# Autodesk Inventor assembly: centre wing
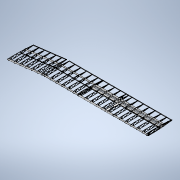
[picture p0: Inventor's stored thumbnail of the model, 180x180]
Saved by Autodesk Inventor 2022 (Build 260153000, 153)
## iProperties
Created: 2021-03-09
Part Number: centre wing
Document SubType Name: Assembly
Designer: Ferdinand Hubbard
Author: Ferdinand Hubbard
## Documents named in this file (20)
- C:\Users\Ferdinand Hubbard\Desktop\solarplane\cad\right wing section.iam
- C:\Users\Ferdinand Hubbard\Desktop\solarplane\cad\tubes\normal tubes\15mm tube.ipt
- C:\Users\Ferdinand Hubbard\Desktop\solarplane\cad\tubes\normal tubes\18mm tube.ipt
- C:\Users\Ferdinand Hubbard\Desktop\solarplane\cad\airfoils\full airfoil\full airfoil blueprint 16 mm.ipt
- C:\Users\Ferdinand Hubbard\Desktop\solarplane\cad\airfoils\full airfoil adjacent to aileron\full adjacent to aileron airfoil 16 mm big hole.ipt
- C:\Users\Ferdinand Hubbard\Desktop\solarplane\cad\airfoils\front half aileron\front half airfoil 19 mm.ipt
- C:\Users\Ferdinand Hubbard\Desktop\solarplane\cad\airfoils\back half aileron\back half aileron airfoil 19mm.ipt
- C:\Users\Ferdinand Hubbard\Desktop\solarplane\cad\tubes\normal tubes\7mm tube.ipt
- C:\Users\Ferdinand Hubbard\Desktop\solarplane\cad\tubes\normal tubes\straight connector aileron spar.ipt
- C:\Users\Ferdinand Hubbard\Desktop\solarplane\cad\airfoils\front half aileron\front half airfoil 16 mm.ipt
- C:\Users\Ferdinand Hubbard\Desktop\solarplane\cad\tubes\normal tubes\angle connector 16 mm.ipt
- C:\Users\Ferdinand Hubbard\Desktop\solarplane\cad\tubes\back aileron tubes\15mm tube.ipt
- C:\Users\Ferdinand Hubbard\Desktop\solarplane\cad\tubes\back aileron tubes\18mm tube.ipt
- C:\Users\Ferdinand Hubbard\Desktop\solarplane\cad\tubes\pre-aileron tubes\angle connector 16 mm.ipt
- C:\Users\Ferdinand Hubbard\Desktop\solarplane\cad\wood spars\wood 5 5 476.ipt
- C:\Users\Ferdinand Hubbard\Desktop\solarplane\cad\wood spars\wood 5 5 478.ipt
- C:\Users\Ferdinand Hubbard\Desktop\solarplane\cad\wood spars\wood 5 5 1459.ipt
- C:\Users\Ferdinand Hubbard\Desktop\solarplane\cad\wood spars\wood 5 5 968.ipt
- C:\Users\Ferdinand Hubbard\Desktop\solarplane\cad\servo mount.ipt
- C:\Users\Ferdinand Hubbard\Desktop\solarplane\cad\aileron arm mount.ipt
## Components (65 placed, 16 different names)
1. angle connector 16 mm:7 — Mate:1, Mate:2, Mate:3, Mate:4, Angle:3
2. angle connector 16 mm:4 — Angle:5, Mate:107
3. 15mm tube:1 — Mate:1, Mate:2, Flush:1, Mate:32, Angle:2, Flush:4, Flush:10
4. 15mm tube:5 — Angle:6, Mate:50, Flush:12, Mate:107, Flush:16
5. 15mm tube:2 — Mate:3, Mate:4, Mate:5, Mate:6, Mate:49, Angle:4
6. 15mm tube:3 — Mate:7, Mate:8, Mate:145
7. 18mm tube:1 — Mate:5, Mate:6, Mate:7, Mate:8, Mate:210
8. full airfoil blueprint 16 mm:1 — Mate:9, Mate:10, Mate:11, Flush:1, Mate:32, Mate:33, Flush:2, Angle:1, Angle:2, Flush:22, Flush:23, Flush:24, Mate:196, Mate:197, Mate:198, Mate:199, Mate:200, Mate:201
9. full airfoil blueprint 16 mm:2 — Mate:9, Mate:10, Mate:11, Mate:15, Mate:16, Mate:17
10. full airfoil blueprint 16 mm:3 — Mate:15, Mate:16, Mate:17
11. full airfoil blueprint 16 mm:4 — Mate:21, Mate:22, Mate:23
12. full airfoil blueprint 16 mm:5 — Mate:21, Mate:22, Mate:23
13. full airfoil blueprint 16 mm:6 — Mate:91, Mate:92
14. 15mm tube:4 — Mate:33, Flush:2, Angle:1, Flush:4, Flush:9
15. full airfoil blueprint 16 mm:7 — Mate:49, Angle:3, Angle:4, Angle:5, Angle:6, Mate:50, Flush:16, Flush:25, Mate:202, Mate:203
16. full airfoil blueprint 16 mm:8
17. full airfoil blueprint 16 mm:9
18. full airfoil blueprint 16 mm:10
19. full airfoil blueprint 16 mm:11 — Mate:93, Flush:11, Mate:104, Mate:105, Mate:106
20. full airfoil blueprint 16 mm:20 — Mate:91, Mate:92, Flush:9, Flush:10
21. full adjacent to aileron airfoil 16 mm big hole:1 — Mate:93, Flush:11, Flush:12, Mate:94, Mate:96, Flush:13, Mate:97, Angle:7, Flush:14, Mate:103, Mate:108, Flush:20, Mate:187, Mate:191, Angle:9
22. front half airfoil 19 mm:1 — Mate:94, Mate:103, Mate:109, Mate:110, Mate:111, Mate:191
23. back half aileron airfoil 19mm:1 — Mate:96, Flush:13, Angle:8, Mate:98, Mate:108, Flush:17, Mate:150, Mate:181, Mate:182
24. 7mm tube:1 — Angle:7, Mate:97, Flush:14, Mate:99, Mate:100, Mate:212
25. 18mm tube:4 — Angle:8, Mate:98, Flush:17, Mate:148, Mate:149, Mate:213
26. straight connector aileron spar:1 — Mate:99, Mate:100, Mate:101, Mate:102
27. 7mm tube:2 — Mate:101, Mate:102, Mate:147
28. full airfoil blueprint 16 mm:21 — Mate:104, Mate:105, Mate:106
29. front half airfoil 19 mm:2 — Mate:109, Mate:110, Mate:111, Mate:115, Mate:116, Mate:117
30. front half airfoil 19 mm:3 — Mate:115, Mate:116, Mate:117
31. front half airfoil 19 mm:4 — Mate:124, Mate:125, Mate:126
32. 18mm tube:3 — Flush:20, Mate:186, Mate:187, Angle:9, Mate:211
33. 15mm tube:6 — Flush:19, Mate:186, Mate:188
34. front half airfoil 19 mm:5 — Mate:124, Mate:125, Mate:126
35. front half airfoil 19 mm:6 — Mate:136, Mate:189, Mate:190
36. front half airfoil 16 mm:1 — Mate:127, Mate:128, Mate:129, Mate:136, Mate:189, Mate:190
37. front half airfoil 16 mm:2 — Mate:127, Mate:128, Mate:129, Mate:133, Mate:134, Mate:135
38. front half airfoil 16 mm:3 — Mate:133, Mate:134, Mate:135
39. front half airfoil 16 mm:4 — Mate:142, Mate:143, Mate:144
40. front half airfoil 16 mm:5 — Mate:142, Mate:143, Mate:144
41. front half airfoil 16 mm:6 — Mate:194, Mate:195
42. full adjacent to aileron airfoil 16 mm big hole:2 — Mate:145, Mate:147, Flush:19, Mate:185, Mate:188, Mate:192, Flush:26, Flush:27, Mate:204, Mate:205, Mate:206, Mate:207
43. 15mm tube:7 — Mate:148, Mate:149, Flush:21
44. back half aileron airfoil 19mm:2 — Mate:150, Mate:151, Mate:152, Mate:153, Mate:181, Mate:182
45. back half aileron airfoil 19mm:3 — Mate:151, Mate:152, Mate:153, Mate:157, Mate:158, Mate:159
46. back half aileron airfoil 19mm:4 — Mate:157, Mate:158, Mate:159
47. back half aileron airfoil 19mm:5 — Mate:169, Mate:170, Mate:171
48. back half aileron airfoil 19mm:6 — Mate:169, Mate:170, Mate:171
49. back half aileron airfoil 19mm:7
50. back half aileron airfoil 19mm:8
51. back half aileron airfoil 19mm:9 — Mate:178, Mate:179, Mate:180
52. back half aileron airfoil 19mm:10 — Mate:178, Mate:179, Mate:180
53. back half aileron airfoil 19mm:11
54. back half aileron airfoil 19mm:12 — Mate:183, Mate:184
55. back half aileron airfoil 19mm:13 — Flush:21, Mate:183, Mate:184, Mate:185, Flush:28, Mate:208, Mate:209
56. front half airfoil 16 mm:7 — Mate:192, Mate:194, Mate:195
57. wood 5 5 476:1 — Flush:24, Mate:200, Mate:201
58. wood 5 5 476:2 — Flush:23, Mate:198, Mate:199
59. wood 5 5 476:3 — Flush:22, Mate:196, Mate:197
60. wood 5 5 478:1 — Flush:25, Mate:202, Mate:203
61. wood 5 5 1459:1 — Flush:27, Mate:206, Mate:207
62. wood 5 5 1459:2 — Flush:26, Mate:204, Mate:205
63. wood 5 5 968:1 — Flush:28, Mate:208, Mate:209
64. servo mount:1 — Mate:210, Mate:211, Mate:214
65. aileron arm mount:1 — Mate:212, Mate:213, Mate:214
## Relationships (188: Mate 158, Flush 21, Angle 9)
- Mate:1: angle connector 16 mm:7 ↔ 15mm tube:1
- Mate:2: angle connector 16 mm:7 ↔ 15mm tube:1
- Mate:3: angle connector 16 mm:7 ↔ 15mm tube:2
- Mate:4: angle connector 16 mm:7 ↔ 15mm tube:2
- Mate:5: 15mm tube:2 ↔ 18mm tube:1
- Mate:6: 15mm tube:2 ↔ 18mm tube:1
- Mate:7: 15mm tube:3 ↔ 18mm tube:1
- Mate:8: 15mm tube:3 ↔ 18mm tube:1
- Mate:9 (80 mm): full airfoil blueprint 16 mm:1 ↔ full airfoil blueprint 16 mm:2
- Mate:10: full airfoil blueprint 16 mm:1 ↔ full airfoil blueprint 16 mm:2
- Mate:11: full airfoil blueprint 16 mm:1 ↔ full airfoil blueprint 16 mm:2
- [Mate] (80 mm): full airfoil blueprint 16 mm:3 ↔ full airfoil blueprint 16 mm:4
- [Mate]: full airfoil blueprint 16 mm:3 ↔ full airfoil blueprint 16 mm:4
- [Mate]: full airfoil blueprint 16 mm:3 ↔ full airfoil blueprint 16 mm:4
- Mate:15: full airfoil blueprint 16 mm:2 ↔ full airfoil blueprint 16 mm:3
- Mate:16: full airfoil blueprint 16 mm:2 ↔ full airfoil blueprint 16 mm:3
- Mate:17 (80 mm): full airfoil blueprint 16 mm:2 ↔ full airfoil blueprint 16 mm:3
- Flush:1 (12 mm): 15mm tube:1 ↔ full airfoil blueprint 16 mm:1
- [Mate] (80 mm): full airfoil blueprint 16 mm:5 ↔ full airfoil blueprint 16 mm:6
- [Mate]: full airfoil blueprint 16 mm:5 ↔ full airfoil blueprint 16 mm:6
- [Mate]: full airfoil blueprint 16 mm:5 ↔ full airfoil blueprint 16 mm:6
- Mate:21 (80 mm): full airfoil blueprint 16 mm:4 ↔ full airfoil blueprint 16 mm:5
- Mate:22: full airfoil blueprint 16 mm:4 ↔ full airfoil blueprint 16 mm:5
- Mate:23: full airfoil blueprint 16 mm:4 ↔ full airfoil blueprint 16 mm:5
- [Mate]: angle connector 16 mm:4 ↔ 15mm tube:4
- [Mate]: angle connector 16 mm:4 ↔ 15mm tube:4
- Mate:32: 15mm tube:1 ↔ full airfoil blueprint 16 mm:1
- Mate:33: full airfoil blueprint 16 mm:1 ↔ 15mm tube:4
- Flush:2 (12 mm): full airfoil blueprint 16 mm:1 ↔ 15mm tube:4
- [Mate] (80 mm): full airfoil blueprint 16 mm:7 ↔ full airfoil blueprint 16 mm:8
- [Mate]: full airfoil blueprint 16 mm:7 ↔ full airfoil blueprint 16 mm:8
- [Mate]: full airfoil blueprint 16 mm:7 ↔ full airfoil blueprint 16 mm:8
- [Mate] (80 mm): full airfoil blueprint 16 mm:9 ↔ full airfoil blueprint 16 mm:10
- [Mate]: full airfoil blueprint 16 mm:9 ↔ full airfoil blueprint 16 mm:10
- [Mate]: full airfoil blueprint 16 mm:9 ↔ full airfoil blueprint 16 mm:10
- [Mate]: full airfoil blueprint 16 mm:8 ↔ full airfoil blueprint 16 mm:9
- [Mate]: full airfoil blueprint 16 mm:8 ↔ full airfoil blueprint 16 mm:9
- [Mate] (80 mm): full airfoil blueprint 16 mm:8 ↔ full airfoil blueprint 16 mm:9
- [Mate] (80 mm): full airfoil blueprint 16 mm:10 ↔ full airfoil blueprint 16 mm:11
- [Mate]: full airfoil blueprint 16 mm:10 ↔ full airfoil blueprint 16 mm:11
- [Mate]: full airfoil blueprint 16 mm:10 ↔ full airfoil blueprint 16 mm:11
- Angle:1 (270 deg): full airfoil blueprint 16 mm:1 ↔ 15mm tube:4
- Angle:2 (270 deg): 15mm tube:1 ↔ full airfoil blueprint 16 mm:1
- Mate:49: 15mm tube:2 ↔ full airfoil blueprint 16 mm:7
- Flush:4: 15mm tube:1 ↔ 15mm tube:4
- Angle:3 (0 deg): angle connector 16 mm:7 ↔ full airfoil blueprint 16 mm:7
- Angle:4 (180 deg): 15mm tube:2 ↔ full airfoil blueprint 16 mm:7
- Angle:5 (0 deg): angle connector 16 mm:4 ↔ full airfoil blueprint 16 mm:7
- Angle:6 (0 deg): 15mm tube:5 ↔ full airfoil blueprint 16 mm:7
- Mate:50: 15mm tube:5 ↔ full airfoil blueprint 16 mm:7
- Mate:91: full airfoil blueprint 16 mm:6 ↔ full airfoil blueprint 16 mm:20
- Mate:92: full airfoil blueprint 16 mm:6 ↔ full airfoil blueprint 16 mm:20
- Flush:9 (12 mm): 15mm tube:4 ↔ full airfoil blueprint 16 mm:20
- Flush:10 (12 mm): 15mm tube:1 ↔ full airfoil blueprint 16 mm:20
- Mate:93: full airfoil blueprint 16 mm:11 ↔ full adjacent to aileron airfoil 16 mm big hole:1
- Flush:11: full airfoil blueprint 16 mm:11 ↔ full adjacent to aileron airfoil 16 mm big hole:1
- Flush:12: 15mm tube:5 ↔ full adjacent to aileron airfoil 16 mm big hole:1
- Mate:94: full adjacent to aileron airfoil 16 mm big hole:1 ↔ front half airfoil 19 mm:1
- Mate:96: full adjacent to aileron airfoil 16 mm big hole:1 ↔ back half aileron airfoil 19mm:1
- Flush:13: full adjacent to aileron airfoil 16 mm big hole:1 ↔ back half aileron airfoil 19mm:1
- Angle:7 (0 deg): full adjacent to aileron airfoil 16 mm big hole:1 ↔ 7mm tube:1
- Mate:97: full adjacent to aileron airfoil 16 mm big hole:1 ↔ 7mm tube:1
- Angle:8 (0 deg): back half aileron airfoil 19mm:1 ↔ 18mm tube:4
- Mate:98: back half aileron airfoil 19mm:1 ↔ 18mm tube:4
- Flush:14 (8 mm): full adjacent to aileron airfoil 16 mm big hole:1 ↔ 7mm tube:1
- Mate:99: 7mm tube:1 ↔ straight connector aileron spar:1
- Mate:100: 7mm tube:1 ↔ straight connector aileron spar:1
- Mate:101: straight connector aileron spar:1 ↔ 7mm tube:2
- Mate:102: straight connector aileron spar:1 ↔ 7mm tube:2
- Mate:103 (12 mm): full adjacent to aileron airfoil 16 mm big hole:1 ↔ front half airfoil 19 mm:1
- Mate:104 (80 mm): full airfoil blueprint 16 mm:11 ↔ full airfoil blueprint 16 mm:21
- Mate:105: full airfoil blueprint 16 mm:11 ↔ full airfoil blueprint 16 mm:21
- Mate:106: full airfoil blueprint 16 mm:11 ↔ full airfoil blueprint 16 mm:21
- Mate:107: angle connector 16 mm:4 ↔ 15mm tube:5
- Flush:16 (22 mm): 15mm tube:5 ↔ full airfoil blueprint 16 mm:7
- Mate:108 (4 mm): full adjacent to aileron airfoil 16 mm big hole:1 ↔ back half aileron airfoil 19mm:1
- Flush:17 (1 mm): back half aileron airfoil 19mm:1 ↔ 18mm tube:4
- Mate:109 (80 mm): front half airfoil 19 mm:1 ↔ front half airfoil 19 mm:2
- Mate:110: front half airfoil 19 mm:1 ↔ front half airfoil 19 mm:2
- Mate:111: front half airfoil 19 mm:1 ↔ front half airfoil 19 mm:2
- [Mate] (80 mm): front half airfoil 19 mm:3 ↔ front half airfoil 19 mm:4
- [Mate]: front half airfoil 19 mm:3 ↔ front half airfoil 19 mm:4
- [Mate]: front half airfoil 19 mm:3 ↔ front half airfoil 19 mm:4
- Mate:115 (80 mm): front half airfoil 19 mm:2 ↔ front half airfoil 19 mm:3
- Mate:116: front half airfoil 19 mm:2 ↔ front half airfoil 19 mm:3
- Mate:117: front half airfoil 19 mm:2 ↔ front half airfoil 19 mm:3
- [Mate]: 18mm tube:3 ↔ 15mm tube:6
- [Mate] (80 mm): front half airfoil 19 mm:5 ↔ front half airfoil 19 mm:6
- [Mate]: front half airfoil 19 mm:5 ↔ front half airfoil 19 mm:6
- [Mate]: front half airfoil 19 mm:5 ↔ front half airfoil 19 mm:6
- Mate:124 (80 mm): front half airfoil 19 mm:4 ↔ front half airfoil 19 mm:5
- Mate:125: front half airfoil 19 mm:4 ↔ front half airfoil 19 mm:5
- Mate:126: front half airfoil 19 mm:4 ↔ front half airfoil 19 mm:5
- Mate:127 (80 mm): front half airfoil 16 mm:1 ↔ front half airfoil 16 mm:2
- Mate:128: front half airfoil 16 mm:1 ↔ front half airfoil 16 mm:2
- Mate:129: front half airfoil 16 mm:1 ↔ front half airfoil 16 mm:2
- [Mate] (80 mm): front half airfoil 16 mm:3 ↔ front half airfoil 16 mm:4
- [Mate]: front half airfoil 16 mm:3 ↔ front half airfoil 16 mm:4
- [Mate]: front half airfoil 16 mm:3 ↔ front half airfoil 16 mm:4
- Mate:133 (80 mm): front half airfoil 16 mm:2 ↔ front half airfoil 16 mm:3
- Mate:134: front half airfoil 16 mm:2 ↔ front half airfoil 16 mm:3
- Mate:135: front half airfoil 16 mm:2 ↔ front half airfoil 16 mm:3
- Mate:136 (80 mm): front half airfoil 19 mm:6 ↔ front half airfoil 16 mm:1
- [Mate] (80 mm): front half airfoil 16 mm:5 ↔ front half airfoil 16 mm:6
- [Mate]: front half airfoil 16 mm:5 ↔ front half airfoil 16 mm:6
- [Mate]: front half airfoil 16 mm:5 ↔ front half airfoil 16 mm:6
- Mate:142 (80 mm): front half airfoil 16 mm:4 ↔ front half airfoil 16 mm:5
- Mate:143: front half airfoil 16 mm:4 ↔ front half airfoil 16 mm:5
- Mate:144: front half airfoil 16 mm:4 ↔ front half airfoil 16 mm:5
- Mate:145: 15mm tube:3 ↔ full adjacent to aileron airfoil 16 mm big hole:2
- Mate:147: 7mm tube:2 ↔ full adjacent to aileron airfoil 16 mm big hole:2
- Mate:148: 18mm tube:4 ↔ 15mm tube:7
- Mate:149: 18mm tube:4 ↔ 15mm tube:7
- Flush:19 (1 mm): 15mm tube:6 ↔ full adjacent to aileron airfoil 16 mm big hole:2
- Mate:150 (80 mm): back half aileron airfoil 19mm:1 ↔ back half aileron airfoil 19mm:2
- Mate:151 (80 mm): back half aileron airfoil 19mm:2 ↔ back half aileron airfoil 19mm:3
- Mate:152: back half aileron airfoil 19mm:2 ↔ back half aileron airfoil 19mm:3
- Mate:153: back half aileron airfoil 19mm:2 ↔ back half aileron airfoil 19mm:3
- [Mate] (80 mm): back half aileron airfoil 19mm:4 ↔ back half aileron airfoil 19mm:5
- [Mate]: back half aileron airfoil 19mm:4 ↔ back half aileron airfoil 19mm:5
- [Mate]: back half aileron airfoil 19mm:4 ↔ back half aileron airfoil 19mm:5
- Mate:157: back half aileron airfoil 19mm:3 ↔ back half aileron airfoil 19mm:4
- Mate:158 (80 mm): back half aileron airfoil 19mm:3 ↔ back half aileron airfoil 19mm:4
- Mate:159: back half aileron airfoil 19mm:3 ↔ back half aileron airfoil 19mm:4
- [Mate] (80 mm): back half aileron airfoil 19mm:6 ↔ back half aileron airfoil 19mm:7
- [Mate]: back half aileron airfoil 19mm:6 ↔ back half aileron airfoil 19mm:7
- [Mate]: back half aileron airfoil 19mm:6 ↔ back half aileron airfoil 19mm:7
- [Mate] (80 mm): back half aileron airfoil 19mm:8 ↔ back half aileron airfoil 19mm:9
- [Mate]: back half aileron airfoil 19mm:8 ↔ back half aileron airfoil 19mm:9
- [Mate]: back half aileron airfoil 19mm:8 ↔ back half aileron airfoil 19mm:9
- [Mate]: back half aileron airfoil 19mm:7 ↔ back half aileron airfoil 19mm:8
- [Mate] (80 mm): back half aileron airfoil 19mm:7 ↔ back half aileron airfoil 19mm:8
- [Mate]: back half aileron airfoil 19mm:7 ↔ back half aileron airfoil 19mm:8
- Mate:169 (80 mm): back half aileron airfoil 19mm:5 ↔ back half aileron airfoil 19mm:6
- Mate:170: back half aileron airfoil 19mm:5 ↔ back half aileron airfoil 19mm:6
- Mate:171: back half aileron airfoil 19mm:5 ↔ back half aileron airfoil 19mm:6
- [Mate] (80 mm): back half aileron airfoil 19mm:11 ↔ back half aileron airfoil 19mm:12
- [Mate]: back half aileron airfoil 19mm:11 ↔ back half aileron airfoil 19mm:12
- [Mate]: back half aileron airfoil 19mm:11 ↔ back half aileron airfoil 19mm:12
- [Mate]: back half aileron airfoil 19mm:10 ↔ back half aileron airfoil 19mm:11
- [Mate] (80 mm): back half aileron airfoil 19mm:10 ↔ back half aileron airfoil 19mm:11
- [Mate]: back half aileron airfoil 19mm:10 ↔ back half aileron airfoil 19mm:11
- Mate:178 (80 mm): back half aileron airfoil 19mm:9 ↔ back half aileron airfoil 19mm:10
- Mate:179: back half aileron airfoil 19mm:9 ↔ back half aileron airfoil 19mm:10
- Mate:180: back half aileron airfoil 19mm:9 ↔ back half aileron airfoil 19mm:10
- Mate:181: back half aileron airfoil 19mm:1 ↔ back half aileron airfoil 19mm:2
- Mate:182: back half aileron airfoil 19mm:1 ↔ back half aileron airfoil 19mm:2
- Flush:21 (1 mm): 15mm tube:7 ↔ back half aileron airfoil 19mm:13
- Mate:183: back half aileron airfoil 19mm:12 ↔ back half aileron airfoil 19mm:13
- Mate:184: back half aileron airfoil 19mm:12 ↔ back half aileron airfoil 19mm:13
- Flush:20 (1 mm): full adjacent to aileron airfoil 16 mm big hole:1 ↔ 18mm tube:3
- Mate:185 (4 mm): full adjacent to aileron airfoil 16 mm big hole:2 ↔ back half aileron airfoil 19mm:13
- Mate:186: 18mm tube:3 ↔ 15mm tube:6
- Mate:187: full adjacent to aileron airfoil 16 mm big hole:1 ↔ 18mm tube:3
- Mate:188: 15mm tube:6 ↔ full adjacent to aileron airfoil 16 mm big hole:2
- Mate:189: front half airfoil 19 mm:6 ↔ front half airfoil 16 mm:1
- Mate:190: front half airfoil 19 mm:6 ↔ front half airfoil 16 mm:1
- Mate:191: full adjacent to aileron airfoil 16 mm big hole:1 ↔ front half airfoil 19 mm:1
- Angle:9 (180 deg): full adjacent to aileron airfoil 16 mm big hole:1 ↔ 18mm tube:3
- Mate:192 (1 mm): full adjacent to aileron airfoil 16 mm big hole:2 ↔ front half airfoil 16 mm:7
- Mate:194: front half airfoil 16 mm:6 ↔ front half airfoil 16 mm:7
- Mate:195: front half airfoil 16 mm:6 ↔ front half airfoil 16 mm:7
- Flush:22: full airfoil blueprint 16 mm:1 ↔ wood 5 5 476:3
- Flush:23: full airfoil blueprint 16 mm:1 ↔ wood 5 5 476:2
- Flush:24: full airfoil blueprint 16 mm:1 ↔ wood 5 5 476:1
- Mate:196: full airfoil blueprint 16 mm:1 ↔ wood 5 5 476:3
- Mate:197: full airfoil blueprint 16 mm:1 ↔ wood 5 5 476:3
- Mate:198: full airfoil blueprint 16 mm:1 ↔ wood 5 5 476:2
- Mate:199: full airfoil blueprint 16 mm:1 ↔ wood 5 5 476:2
- Mate:200: full airfoil blueprint 16 mm:1 ↔ wood 5 5 476:1
- Mate:201: full airfoil blueprint 16 mm:1 ↔ wood 5 5 476:1
- Flush:25: full airfoil blueprint 16 mm:7 ↔ wood 5 5 478:1
- Mate:202: full airfoil blueprint 16 mm:7 ↔ wood 5 5 478:1
- Mate:203: full airfoil blueprint 16 mm:7 ↔ wood 5 5 478:1
- Flush:26: full adjacent to aileron airfoil 16 mm big hole:2 ↔ wood 5 5 1459:2
- Flush:27: full adjacent to aileron airfoil 16 mm big hole:2 ↔ wood 5 5 1459:1
- Mate:204: full adjacent to aileron airfoil 16 mm big hole:2 ↔ wood 5 5 1459:2
- Mate:205: full adjacent to aileron airfoil 16 mm big hole:2 ↔ wood 5 5 1459:2
- Mate:206: full adjacent to aileron airfoil 16 mm big hole:2 ↔ wood 5 5 1459:1
- Mate:207: full adjacent to aileron airfoil 16 mm big hole:2 ↔ wood 5 5 1459:1
- Flush:28: back half aileron airfoil 19mm:13 ↔ wood 5 5 968:1
- Mate:208: back half aileron airfoil 19mm:13 ↔ wood 5 5 968:1
- Mate:209: back half aileron airfoil 19mm:13 ↔ wood 5 5 968:1
- Mate:210: 18mm tube:1 ↔ servo mount:1
- Mate:211: 18mm tube:3 ↔ servo mount:1
- Mate:212: 7mm tube:1 ↔ aileron arm mount:1
- Mate:213: 18mm tube:4 ↔ aileron arm mount:1
- Mate:214 (16.7 mm): servo mount:1 ↔ aileron arm mount:1
## Named parameters: d220_d217 = 80 mm, d221_d218 = 0 mm, d222_d219 = 0 mm, d227_d220_d217 = 80 mm, d228_d221_d218 = 0 mm, d229_d222_d219 = 0 mm, d233_d209 = 0 mm, d234_d210 = 0 mm, d244_d217 = 80 mm, d245_d218 = 0 mm, d246_d219 = 0 mm, d247_d220_d217 = 80 mm, d248_d221_d218 = 0 mm, d249_d222_d219 = 0 mm, d250_d223 = 0 mm, d251_d224 = 0 mm, d252_d225 = 80 mm, d256_d230 = 80 mm, d257_d231 = 0 mm, d258_d232 = 0 mm, d355_d352 = 80 mm, d356_d353 = 0 mm, d357_d354 = 0 mm, d363_d215 = 0 mm, d367_d355_d352 = 80 mm, d368_d356_d353 = 0 mm, d369_d357_d354 = 0 mm, d376_d373 = 80 mm, d377_d374 = 0 mm, d378_d375 = 0 mm, d385_d376_d373 = 80 mm, d386_d377_d374 = 0 mm, d387_d378_d375 = 0 mm, d401_d398 = 80 mm, d402_d399 = 0 mm, d403_d400 = 0 mm, d407_d398 = 80 mm, d408_d399 = 0 mm, d409_d400 = 0 mm, d410_d401_d398 = 80 mm, d411_d402_d399 = 0 mm, d412_d403_d400 = 0 mm, d413_d404 = 0 mm, d414_d405 = 80 mm, d415_d406 = 0 mm, d419_d410_d401_d398 = 80 mm, d420_d411_d402_d399 = 0 mm, d421_d412_d403_d400 = 0 mm, d422_d413_d404 = 0 mm, d423_d414_d405 = 80 mm, d424_d415_d406 = 0 mm
